# Autodesk Inventor assembly: Top Braces
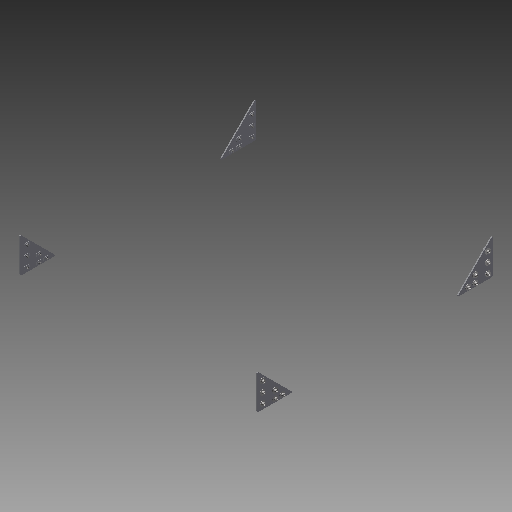
[picture p0: Inventor's stored thumbnail of the model, 512x512]
Saved by Autodesk Inventor 2018 (Build 220112000, 112)
## iProperties
Created: 2016-08-02
Part Number: Top Braces
Document SubType Name: Assembly
Designer: User
Author: User
## Documents named in this file (6)
- C:\Users\Dan\OneDrive\SL-Inventor\The Beast v1.2 PackandGo\Workspaces\Workspace\Top Braces.iam
- C:\Users\Dan\OneDrive\SL-Inventor\The Beast v1.2 PackandGo\Workspaces\Workspace\Side Brace.ipt
- C:\Users\Dan\OneDrive\SL-Inventor\The Beast v1.2 PackandGo\Workspaces\Workspace\Side Brace_MIR.ipt
- C:\Users\Dan\OneDrive\SL-Inventor\The Beast v1.2 PackandGo\Workspaces\Workspace\Side Brace_MIR1.ipt
- C:\Users\Dan\OneDrive\SL-Inventor\The Beast v1.2 PackandGo\Workspaces\Workspace\Side Brace_MIR_MIR.ipt
- C:\Users\Dan\OneDrive\SL-Inventor\The Beast v1.2 PackandGo\Workspaces\Workspace\BoltandTee.iam
## Components (28 placed, 5 different names)
1. Side Brace:1
2. Side Brace_MIR:1
3. Side Brace_MIR1:1
4. Side Brace_MIR_MIR:1 — Insert:33
5. BoltandTee:1 [sub-assembly]
6. BoltandTee:2 [sub-assembly]
7. BoltandTee:3 [sub-assembly]
8. BoltandTee:4 [sub-assembly]
9. BoltandTee:5 [sub-assembly]
10. BoltandTee:6 [sub-assembly]
11. BoltandTee:7 [sub-assembly]
12. BoltandTee:8 [sub-assembly]
13. BoltandTee:9 [sub-assembly]
14. BoltandTee:10 [sub-assembly]
15. BoltandTee:11 [sub-assembly]
16. BoltandTee:17 [sub-assembly]
17. BoltandTee:18 [sub-assembly]
18. BoltandTee:19 [sub-assembly]
19. BoltandTee:20 [sub-assembly]
20. BoltandTee:21 [sub-assembly]
21. BoltandTee:22 [sub-assembly]
22. BoltandTee:28 [sub-assembly]
23. BoltandTee:29 [sub-assembly]
24. BoltandTee:30 [sub-assembly]
25. BoltandTee:31 [sub-assembly]
26. BoltandTee:32 [sub-assembly]
27. BoltandTee:33 [sub-assembly]
28. BoltandTee:34 [sub-assembly] — Insert:33
## Relationships (25: Insert 23, Mate 2)
- [Mate]: Side Brace_MIR_MIR:1 ↔ BoltandTee:1
- [Mate]: Side Brace_MIR_MIR:1 ↔ BoltandTee:1
- [Insert]: Side Brace_MIR:1 ↔ BoltandTee:3
- [Insert]: Side Brace_MIR:1 ↔ BoltandTee:4
- [Insert]: Side Brace_MIR:1 ↔ BoltandTee:5
- [Insert]: Side Brace_MIR:1 ↔ BoltandTee:7
- [Insert]: Side Brace_MIR:1 ↔ BoltandTee:6
- [Insert]: Side Brace_MIR:1 ↔ BoltandTee:8
- [Insert]: Side Brace_MIR_MIR:1 ↔ BoltandTee:2
- [Insert]: Side Brace_MIR_MIR:1 ↔ BoltandTee:9
- [Insert]: Side Brace_MIR_MIR:1 ↔ BoltandTee:11
- [Insert]: Side Brace_MIR_MIR:1 ↔ BoltandTee:10
- [Insert]: Side Brace:1 ↔ BoltandTee:17
- [Insert]: Side Brace:1 ↔ BoltandTee:18
- [Insert]: Side Brace:1 ↔ BoltandTee:19
- [Insert]: Side Brace:1 ↔ BoltandTee:20
- [Insert]: Side Brace:1 ↔ BoltandTee:21
- [Insert]: Side Brace:1 ↔ BoltandTee:22
- [Insert]: Side Brace_MIR1:1 ↔ BoltandTee:31
- [Insert]: Side Brace_MIR1:1 ↔ BoltandTee:32
- [Insert]: Side Brace_MIR1:1 ↔ BoltandTee:33
- [Insert]: Side Brace_MIR1:1 ↔ BoltandTee:30
- [Insert]: Side Brace_MIR1:1 ↔ BoltandTee:29
- [Insert]: Side Brace_MIR1:1 ↔ BoltandTee:28
- Insert:33: Side Brace_MIR_MIR:1 ↔ BoltandTee:34
